# Autodesk Inventor assembly: 組立図
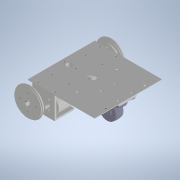
[picture p0: Inventor's stored thumbnail of the model, 180x180]
Saved by Autodesk Inventor 2021 (Build 250183000, 183)
## iProperties
Created: 2020-11-01
Part Number: 組立図
Document SubType Name: Assembly
Designer: ryusei
Author: ryusei
## Documents named in this file (18)
- C:\Users\ryusei\Documents\Inventor\robot_design_2020\組立図.iam
- C:\Users\ryusei\Documents\Inventor\robot_design_2020\RD002_フレーム.ipt
- C:\Users\ryusei\Documents\Inventor\robot_design_2020\RD004_スペーサ.ipt
- C:\Users\ryusei\Documents\Inventor\robot_design_2020\RD003_キャスタ420G-R32.ipt
- C:\Users\ryusei\Documents\Inventor\robot_design_2020\RD005_ペンホルダ.ipt
- C:\Users\ryusei\Documents\Inventor\robot_design_2020\RD006_ギアボックス(左).ipt
- C:\Users\ryusei\Documents\Inventor\robot_design_2020\RD007_ギアボックス(右).ipt
- C:\Users\ryusei\Documents\Inventor\robot_design_2020\RD008_モータ(DMN29).ipt
- C:\Users\ryusei\Documents\Inventor\robot_design_2020\RD009_ギアDS0.5-12.ipt
- C:\Users\ryusei\Documents\Inventor\robot_design_2020\RD014_ストッパKC18.ipt
- C:\Users\ryusei\Documents\Inventor\robot_design_2020\RD015_シャフト.ipt
- C:\Users\ryusei\Documents\Inventor\robot_design_2020\RD018_ワッシャ.ipt
- C:\Users\ryusei\Documents\Inventor\robot_design_2020\RD017_ブッシュ80F- 0305改.ipt
- C:\Users\ryusei\Documents\Inventor\robot_design_2020\RD010_ギアDS0.5-80.ipt
- C:\Users\ryusei\Documents\Inventor\robot_design_2020\RD011_ギア用ブッシュ.ipt
- C:\Users\ryusei\Documents\Inventor\robot_design_2020\RD012_ホイール.ipt
- C:\Users\ryusei\Documents\Inventor\robot_design_2020\RD016_ブッシュ80F- 0305.ipt
- C:\Users\ryusei\Documents\Inventor\robot_design_2020\RD013_オーリング.ipt
## Components (30 placed, 17 different names)
1. RD002_フレーム:1 — 挿入:1, 挿入:2, 挿入:5, 挿入:6, 挿入:7, メイト:1, 挿入:8, 挿入:9
2. RD004_スペーサ:1 — 挿入:1, 挿入:2, 挿入:3, 挿入:4
3. RD003_キャスタ420G-R32:1 — 挿入:3, 挿入:4
4. RD005_ペンホルダ:1 — 挿入:5, 挿入:6
5. RD006_ギアボックス(左):1 — 挿入:7, メイト:1, 挿入:12, 挿入:13, 挿入:17, 挿入:22
6. RD007_ギアボックス(右):1 — 挿入:8, 挿入:9, 挿入:10, 挿入:11, 挿入:16, 挿入:21
7. RD008_モータ(DMN29):1 — 挿入:12, 挿入:13, 挿入:14
8. RD008_モータ(DMN29):2 — 挿入:10, 挿入:11, 挿入:18
9. RD009_ギアDS0.5-12:1 — 挿入:18
10. RD009_ギアDS0.5-12:2 — 挿入:14
11. RD014_ストッパKC18:1 — 挿入:16, 挿入:19
12. RD014_ストッパKC18:2 — 挿入:17, 挿入:20
13. RD015_シャフト:1 — 挿入:20
14. RD015_シャフト:2 — 挿入:19
15. RD018_ワッシャ:1 — 挿入:21, 挿入:24
16. RD018_ワッシャ:2 — 挿入:22, 挿入:23
17. RD017_ブッシュ80F- 0305改:1 — 挿入:24, 挿入:27
18. RD017_ブッシュ80F- 0305改:2 — 挿入:23, 挿入:28
19. RD010_ギアDS0.5-80:1 — 挿入:26, 挿入:35
20. RD010_ギアDS0.5-80:2 — 挿入:25, 挿入:36
21. RD011_ギア用ブッシュ:1 — 挿入:25, 挿入:27, 挿入:32
22. RD011_ギア用ブッシュ:2 — 挿入:26, 挿入:28, 挿入:31
23. RD012_ホイール:1 — 挿入:29, 挿入:35, メイト:3, 正接:2
24. RD012_ホイール:2 — 挿入:30, 挿入:36, メイト:2, 正接:1
25. RD016_ブッシュ80F- 0305:1 — 挿入:29, 挿入:31, 挿入:34
26. RD016_ブッシュ80F- 0305:2 — 挿入:30, 挿入:32, 挿入:33
27. RD014_ストッパKC18:3 — 挿入:34
28. RD014_ストッパKC18:4 — 挿入:33
29. RD013_オーリング:1 — メイト:3, 正接:2
30. RD013_オーリング:2 — メイト:2, 正接:1
## Relationships (40: Insert 35, Mate 3, Tangent 2)
- 挿入:1 [Insert]: RD002_フレーム:1 ↔ RD004_スペーサ:1
- 挿入:2 [Insert]: RD002_フレーム:1 ↔ RD004_スペーサ:1
- 挿入:3 [Insert]: RD004_スペーサ:1 ↔ RD003_キャスタ420G-R32:1
- 挿入:4 [Insert]: RD004_スペーサ:1 ↔ RD003_キャスタ420G-R32:1
- 挿入:5 [Insert]: RD002_フレーム:1 ↔ RD005_ペンホルダ:1
- 挿入:6 [Insert]: RD002_フレーム:1 ↔ RD005_ペンホルダ:1
- 挿入:7 [Insert]: RD002_フレーム:1 ↔ RD006_ギアボックス(左):1
- メイト:1 [Mate]: RD002_フレーム:1 ↔ RD006_ギアボックス(左):1
- 挿入:8 [Insert]: RD002_フレーム:1 ↔ RD007_ギアボックス(右):1
- 挿入:9 [Insert]: RD002_フレーム:1 ↔ RD007_ギアボックス(右):1
- 挿入:10 [Insert]: RD007_ギアボックス(右):1 ↔ RD008_モータ(DMN29):2
- 挿入:11 [Insert]: RD007_ギアボックス(右):1 ↔ RD008_モータ(DMN29):2
- 挿入:12 [Insert]: RD006_ギアボックス(左):1 ↔ RD008_モータ(DMN29):1
- 挿入:13 [Insert]: RD006_ギアボックス(左):1 ↔ RD008_モータ(DMN29):1
- 挿入:14 [Insert]: RD008_モータ(DMN29):1 ↔ RD009_ギアDS0.5-12:2
- 挿入:16 [Insert]: RD007_ギアボックス(右):1 ↔ RD014_ストッパKC18:1
- 挿入:17 [Insert]: RD006_ギアボックス(左):1 ↔ RD014_ストッパKC18:2
- 挿入:18 [Insert]: RD008_モータ(DMN29):2 ↔ RD009_ギアDS0.5-12:1
- 挿入:19 [Insert]: RD014_ストッパKC18:1 ↔ RD015_シャフト:2
- 挿入:20 [Insert]: RD014_ストッパKC18:2 ↔ RD015_シャフト:1
- 挿入:21 [Insert]: RD007_ギアボックス(右):1 ↔ RD018_ワッシャ:1
- 挿入:22 [Insert]: RD006_ギアボックス(左):1 ↔ RD018_ワッシャ:2
- 挿入:23 [Insert]: RD018_ワッシャ:2 ↔ RD017_ブッシュ80F- 0305改:2
- 挿入:24 [Insert]: RD018_ワッシャ:1 ↔ RD017_ブッシュ80F- 0305改:1
- 挿入:25 [Insert]: RD010_ギアDS0.5-80:2 ↔ RD011_ギア用ブッシュ:1
- 挿入:26 [Insert]: RD010_ギアDS0.5-80:1 ↔ RD011_ギア用ブッシュ:2
- 挿入:27 [Insert]: RD017_ブッシュ80F- 0305改:1 ↔ RD011_ギア用ブッシュ:1
- 挿入:28 [Insert]: RD017_ブッシュ80F- 0305改:2 ↔ RD011_ギア用ブッシュ:2
- 挿入:29 [Insert]: RD012_ホイール:1 ↔ RD016_ブッシュ80F- 0305:1
- 挿入:30 [Insert]: RD012_ホイール:2 ↔ RD016_ブッシュ80F- 0305:2
- 挿入:31 [Insert]: RD011_ギア用ブッシュ:2 ↔ RD016_ブッシュ80F- 0305:1
- 挿入:32 [Insert]: RD011_ギア用ブッシュ:1 ↔ RD016_ブッシュ80F- 0305:2
- 挿入:33 [Insert]: RD016_ブッシュ80F- 0305:2 ↔ RD014_ストッパKC18:4
- 挿入:34 [Insert]: RD016_ブッシュ80F- 0305:1 ↔ RD014_ストッパKC18:3
- 挿入:35 [Insert]: RD010_ギアDS0.5-80:1 ↔ RD012_ホイール:1
- 挿入:36 [Insert]: RD010_ギアDS0.5-80:2 ↔ RD012_ホイール:2
- メイト:2 [Mate]: RD012_ホイール:2 ↔ RD013_オーリング:2
- 正接:1 [Tangent]: RD012_ホイール:2 ↔ RD013_オーリング:2
- メイト:3 [Mate]: RD012_ホイール:1 ↔ RD013_オーリング:1
- 正接:2 [Tangent]: RD012_ホイール:1 ↔ RD013_オーリング:1
